# Autodesk Inventor assembly: Leg_joint_roll_pitch
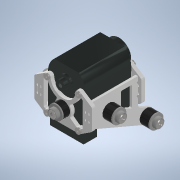
[picture p0: Inventor's stored thumbnail of the model, 180x180]
Saved by Autodesk Inventor 2020.4 (Build 244396000, 396)
## iProperties
Part Number: Leg_joint_roll_pitch
Document SubType Name: Assembly
Designer: Masato Kubotera
Mass: 155.537 g
Surface Area: 333.044 cm^2
Volume: 75.5065 cm^3
Density: 2.05992 g/cm^3
Author: Masato Kubotera
## Documents named in this file (16)
- C:\Users\Masato\Documents\Inventor\CIT Brains_Inventor\OpenPlatform_ver3_0（ワッシャ変更）\LowerBody\Leg_joit\Leg_joint_roll_pitch.iam
- C:\Users\Masato\Documents\Inventor\CIT Brains_Inventor\OpenPlatform_ver3_0（ワッシャ変更）\LowerBody\Leg_joit\Leg_joint_pitch_frame.ipt
- C:\Users\Masato\Documents\Inventor\CIT Brains_Inventor\OpenPlatform_ver3_0（ワッシャ変更）\LowerBody\Leg_joit\Leg_joint_roll_frame.ipt
- C:\Users\Masato\Documents\Inventor\CIT Brains_Inventor\OpenPlatform_ver3_0（ワッシャ変更）\Ready_Made\B3M11xx.ipt
- C:\Users\Masato\Documents\Inventor\CIT Brains_Inventor\OpenPlatform_ver3_0（ワッシャ変更）\Ready_Made\SLSBF6-39_5-M3-N3.ipt
- C:\Users\Masato\Documents\Inventor\CIT Brains_Inventor\OpenPlatform_ver3_0（ワッシャ変更）\Ready_Made\UUW-0312-10BH.ipt
- C:\Users\Masato\Documents\Inventor\CIT Brains_Inventor\OpenPlatform_ver3_0（ワッシャ変更）\Ready_Made\S3-07-3W.ipt
- C:\Users\Masato\Documents\Inventor\CIT Brains_Inventor\OpenPlatform_ver3_0（ワッシャ変更）\Ready_Made\BRU-311S.ipt
- C:\Users\Masato\Documents\Inventor\CIT Brains_Inventor\OpenPlatform_ver3_0（ワッシャ変更）\Ready_Made\ARU-309S.ipt
- C:\Users\Masato\Documents\Inventor\CIT Brains_Inventor\OpenPlatform_ver3_0（ワッシャ変更）\Ready_Made\Screw\M3-6.ipt
- C:\Users\Masato\Documents\Inventor\CIT Brains_Inventor\OpenPlatform_ver3_0（ワッシャ変更）\Ready_Made\Screw\M2_6-20.ipt
- C:\Users\Masato\Documents\Inventor\CIT Brains_Inventor\OpenPlatform_ver3_0（ワッシャ変更）\Ready_Made\Screw\M2_6-15.ipt
- C:\Users\Masato\Documents\Inventor\CIT Brains_Inventor\OpenPlatform_ver3_0（ワッシャ変更）\Ready_Made\80F-0603.ipt
- C:\Users\Masato\Documents\Inventor\CIT Brains_Inventor\OpenPlatform_ver3_0（ワッシャ変更）\Ready_Made\CC-0612-15B.ipt
- C:\Users\Masato\Documents\Inventor\CIT Brains_Inventor\OpenPlatform_ver3_0（ワッシャ変更）\Ready_Made\CC-0612-50B.ipt
- C:\Users\Masato\Documents\Inventor\CIT Brains_Inventor\OpenPlatform_ver3_0（ワッシャ変更）\Ready_Made\CC-0612-30B.ipt
## Components (48 placed, 15 different names)
1. Leg_joint_pitch_frame:1 — メイト:2, フラッシュ:1, 挿入:11, 挿入:27, 挿入:28, 挿入:45
2. Leg_joint_pitch_frame:2 — メイト:3, メイト:4, フラッシュ:2, 挿入:12, 挿入:25, 挿入:26, 挿入:46, フラッシュ:1
3. Leg_joint_roll_frame:1 — 挿入:3, 挿入:4, 挿入:5, 挿入:6, メイト:2, メイト:3, メイト:4, フラッシュ:2, 挿入:81, 挿入:104, 挿入:106, 挿入:107, 挿入:108, 挿入:109
4. Leg_joint_roll_frame:2 — 挿入:7, 挿入:8, 挿入:9, 挿入:10, 挿入:55, 挿入:105, 挿入:110, 挿入:111, 挿入:112, 挿入:113
5. B3M11xx:1 — 挿入:3, 挿入:4, 挿入:5, 挿入:6, 挿入:7, 挿入:8, 挿入:9, 挿入:10, フラッシュ:6, メイト:8, メイト:10
6. SLSBF6-39_5-M3-N3:1 — 挿入:11, 挿入:12
7. UUW-0312-10BH:1 — 挿入:27, 挿入:100, 挿入:124
8. UUW-0312-10BH:2 — 挿入:28, 挿入:101, 挿入:125
9. UUW-0312-10BH:3 — 挿入:25, 挿入:99, 挿入:126
10. UUW-0312-10BH:4 — 挿入:26, 挿入:98, 挿入:127
11. S3-07-3W:1 — 挿入:45
12. S3-07-3W:2 — 挿入:46
13. UUW-0312-10BH:5 — 挿入:55, 挿入:103, 挿入:121
14. UUW-0312-10BH:6 — 挿入:81, 挿入:102, 挿入:120
15. BRU-311S:1 — 挿入:99
16. BRU-311S:2 — 挿入:98
17. BRU-311S:3 — 挿入:101
18. BRU-311S:4 — 挿入:100
19. ARU-309S:1 — 挿入:102
20. ARU-309S:2 — 挿入:103
21. M3-6:1 — 挿入:104
22. M3-6:2 — 挿入:105
23. M2_6-20:1 — 挿入:106
24. M2_6-20:2 — 挿入:107
25. M2_6-20:3 — 挿入:108
26. M2_6-20:4 — 挿入:109
27. M2_6-15:1 — 挿入:110
28. M2_6-15:2 — 挿入:111
29. M2_6-15:3 — 挿入:112
30. M2_6-15:4 — 挿入:113
31. 80F-0603:1 — 挿入:123
32. 80F-0603:2 — 挿入:122
33. 80F-0603:3 — 挿入:130
34. 80F-0603:4 — 挿入:131
35. 80F-0603:5 — 挿入:129
36. 80F-0603:6 — 挿入:128
37. CC-0612-15B:1 — 挿入:114, 挿入:124
38. CC-0612-15B:2 — 挿入:115, 挿入:125
39. CC-0612-15B:3 — 挿入:116, 挿入:127
40. CC-0612-15B:4 — 挿入:117, 挿入:126
41. CC-0612-15B:5 — 挿入:118, 挿入:120
42. CC-0612-15B:6 — 挿入:119, 挿入:121
43. CC-0612-50B:1 — 挿入:114, 挿入:130
44. CC-0612-50B:2 — 挿入:115, 挿入:131
45. CC-0612-50B:3 — 挿入:116, 挿入:128
46. CC-0612-50B:4 — 挿入:117, 挿入:129
47. CC-0612-30B:1 — 挿入:118, 挿入:123
48. CC-0612-30B:2 — 挿入:119, 挿入:122
## Relationships (60: Insert 52, Mate 5, Flush 3)
- 挿入:3 [Insert]: Leg_joint_roll_frame:1 ↔ B3M11xx:1
- 挿入:4 [Insert]: Leg_joint_roll_frame:1 ↔ B3M11xx:1
- 挿入:5 [Insert]: Leg_joint_roll_frame:1 ↔ B3M11xx:1
- 挿入:6 [Insert]: Leg_joint_roll_frame:1 ↔ B3M11xx:1
- 挿入:7 [Insert]: Leg_joint_roll_frame:2 ↔ B3M11xx:1
- 挿入:8 [Insert]: Leg_joint_roll_frame:2 ↔ B3M11xx:1
- 挿入:9 [Insert]: Leg_joint_roll_frame:2 ↔ B3M11xx:1
- 挿入:10 [Insert]: Leg_joint_roll_frame:2 ↔ B3M11xx:1
- メイト:2 [Mate] (0.01 mm): Leg_joint_pitch_frame:1 ↔ Leg_joint_roll_frame:1
- フラッシュ:1 [Flush]: Leg_joint_pitch_frame:1 ↔ Leg_joint_pitch_frame:2
- メイト:3 [Mate] (0.01 mm): Leg_joint_pitch_frame:2 ↔ Leg_joint_roll_frame:1
- メイト:4 [Mate] (0.01 mm): Leg_joint_pitch_frame:2 ↔ Leg_joint_roll_frame:1
- フラッシュ:2 [Flush]: Leg_joint_pitch_frame:2 ↔ Leg_joint_roll_frame:1
- 挿入:11 [Insert]: Leg_joint_pitch_frame:1 ↔ SLSBF6-39_5-M3-N3:1
- 挿入:12 [Insert]: Leg_joint_pitch_frame:2 ↔ SLSBF6-39_5-M3-N3:1
- 挿入:25 [Insert]: Leg_joint_pitch_frame:2 ↔ UUW-0312-10BH:3
- 挿入:26 [Insert]: Leg_joint_pitch_frame:2 ↔ UUW-0312-10BH:4
- 挿入:27 [Insert]: Leg_joint_pitch_frame:1 ↔ UUW-0312-10BH:1
- 挿入:28 [Insert]: Leg_joint_pitch_frame:1 ↔ UUW-0312-10BH:2
- フラッシュ:6 [Flush]: B3M11xx:1
- メイト:8 [Mate]: B3M11xx:1
- 挿入:45 [Insert]: Leg_joint_pitch_frame:1 ↔ S3-07-3W:1
- 挿入:46 [Insert]: Leg_joint_pitch_frame:2 ↔ S3-07-3W:2
- 挿入:55 [Insert]: Leg_joint_roll_frame:2 ↔ UUW-0312-10BH:5
- メイト:10 [Mate]: B3M11xx:1
- 挿入:81 [Insert]: Leg_joint_roll_frame:1 ↔ UUW-0312-10BH:6
- 挿入:98 [Insert]: UUW-0312-10BH:4 ↔ BRU-311S:2
- 挿入:99 [Insert]: UUW-0312-10BH:3 ↔ BRU-311S:1
- 挿入:100 [Insert]: UUW-0312-10BH:1 ↔ BRU-311S:4
- 挿入:101 [Insert]: UUW-0312-10BH:2 ↔ BRU-311S:3
- 挿入:102 [Insert]: UUW-0312-10BH:6 ↔ ARU-309S:1
- 挿入:103 [Insert]: UUW-0312-10BH:5 ↔ ARU-309S:2
- 挿入:104 [Insert]: Leg_joint_roll_frame:1 ↔ M3-6:1
- 挿入:105 [Insert]: Leg_joint_roll_frame:2 ↔ M3-6:2
- 挿入:106 [Insert]: Leg_joint_roll_frame:1 ↔ M2_6-20:1
- 挿入:107 [Insert]: Leg_joint_roll_frame:1 ↔ M2_6-20:2
- 挿入:108 [Insert]: Leg_joint_roll_frame:1 ↔ M2_6-20:3
- 挿入:109 [Insert]: Leg_joint_roll_frame:1 ↔ M2_6-20:4
- 挿入:110 [Insert]: Leg_joint_roll_frame:2 ↔ M2_6-15:1
- 挿入:111 [Insert]: Leg_joint_roll_frame:2 ↔ M2_6-15:2
- 挿入:112 [Insert]: Leg_joint_roll_frame:2 ↔ M2_6-15:3
- 挿入:113 [Insert]: Leg_joint_roll_frame:2 ↔ M2_6-15:4
- 挿入:114 [Insert]: CC-0612-15B:1 ↔ CC-0612-50B:1
- 挿入:115 [Insert]: CC-0612-15B:2 ↔ CC-0612-50B:2
- 挿入:116 [Insert]: CC-0612-15B:3 ↔ CC-0612-50B:3
- 挿入:117 [Insert]: CC-0612-15B:4 ↔ CC-0612-50B:4
- 挿入:118 [Insert]: CC-0612-15B:5 ↔ CC-0612-30B:1
- 挿入:119 [Insert]: CC-0612-15B:6 ↔ CC-0612-30B:2
- 挿入:120 [Insert]: UUW-0312-10BH:6 ↔ CC-0612-15B:5
- 挿入:121 [Insert]: UUW-0312-10BH:5 ↔ CC-0612-15B:6
- 挿入:122 [Insert]: 80F-0603:2 ↔ CC-0612-30B:2
- 挿入:123 [Insert]: 80F-0603:1 ↔ CC-0612-30B:1
- 挿入:124 [Insert]: UUW-0312-10BH:1 ↔ CC-0612-15B:1
- 挿入:125 [Insert]: UUW-0312-10BH:2 ↔ CC-0612-15B:2
- 挿入:126 [Insert]: UUW-0312-10BH:3 ↔ CC-0612-15B:4
- 挿入:127 [Insert]: UUW-0312-10BH:4 ↔ CC-0612-15B:3
- 挿入:128 [Insert]: 80F-0603:6 ↔ CC-0612-50B:3
- 挿入:129 [Insert]: 80F-0603:5 ↔ CC-0612-50B:4
- 挿入:130 [Insert]: 80F-0603:3 ↔ CC-0612-50B:1
- 挿入:131 [Insert]: 80F-0603:4 ↔ CC-0612-50B:2
